# Autodesk Inventor assembly: NCJ2D10-200
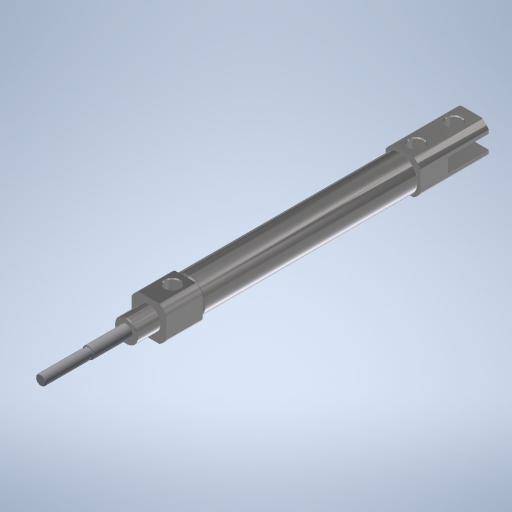
[picture p0: Inventor's stored thumbnail of the model, 512x512]
Saved by Autodesk Inventor 2023 (Build 270158000, 158)
## iProperties
Company: Bots 'n' Stuff
Created: 2006-09-22
Part Number: NCJ2D10-200
Vendor: SMC Corporation
Document SubType Name: Assembly
Designer: Jordan Kiesel
Catalog Web Link: http://smcpneumatics.com/NCJ2D10-200.html
Mass: 74.3314 g
Surface Area: 91.0681 cm^2
Volume: 9.29142 cm^3
Density: 8 g/cm^3
Title: Cylinder, Bi-directional
Author: Jordan Kiesel
## Documents named in this file (3)
- C:\Users\aaron\Documents\Inventor\Spin Up\library\Motion\Pneumatics\Cylinder, Bi-directional.iam
- C:\Users\aaron\Documents\Inventor\Spin Up\library\Motion\Pneumatics\Reference Parts\Cylinder, Bi-directional\NCJ2-Body 10D.ipt
- C:\Users\aaron\Documents\Inventor\Spin Up\library\Motion\Pneumatics\Reference Parts\Cylinder, Bi-directional\NCJ2-Rod 10.ipt
## Components (2 placed, 2 different names)
1. NCJ2-Body 10D:1 — Insert:1
2. NCJ2-Rod 10:1 — Insert:1
## Relationships (1: Insert 1)
- Insert:1: NCJ2-Body 10D:1 ↔ NCJ2-Rod 10:1
